# Autodesk Inventor assembly: Pass_Hang_subass
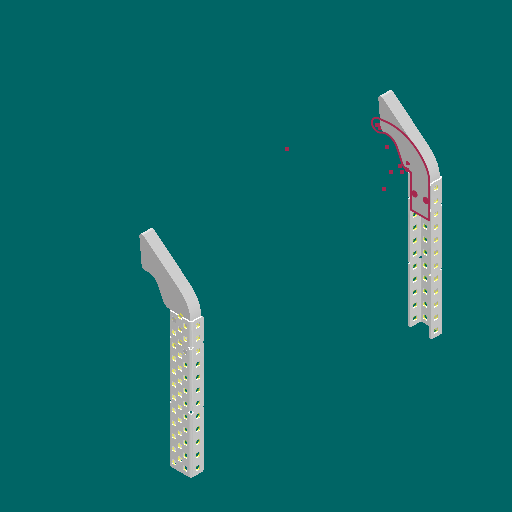
[picture p0: Inventor's stored thumbnail of the model, 512x512]
Saved by Autodesk Inventor 2025.2 (Build 292293000, 293)
## iProperties
Created: 2025-01-10
Part Number: Pass_Hang_subass
Document SubType Name: Assembly
Designer: Juanl
Author: Juanl
## Documents named in this file (4)
- C:\Users\colli\Documents\GitHub\ATUM-V5RC-High-Stakes-CAD\Robot\Subassemblies\Pass_Hang_subass.iam
- C:\Users\colli\Documents\GitHub\ATUM-V5RC-High-Stakes-CAD\Protobot\Pass_Hang_Hook.ipt
- C:\Users\colli\Documents\GitHub\ATUM-V5RC-High-Stakes-CAD\Protobot\Pass_Hang_Hook_MIR.ipt
- C:\Users\colli\Documents\GitHub\ATUM-V5RC-High-Stakes-CAD\VEX-CAD-Inventor\Structure\C Channel\Aluminum 1x2x1\Alu C 1x2x1x12.ipt
## Components (4 placed, 3 different names)
1. Pass_Hang_Hook:1 — Mate:3, Mate:4, Mate:5
2. Pass_Hang_Hook_MIR:1 — Mate:1, Mate:2, Mate:5
3. Alu C 1x2x1x12:2 — Flush:1, Mate:3, Mate:4, Mate:6
4. Alu C 1x2x1x12:1 — Flush:1, Mate:1, Mate:2, Mate:6
## Relationships (7: Mate 6, Flush 1)
- Flush:1: Alu C 1x2x1x12:2 ↔ Alu C 1x2x1x12:1
- Mate:1: Pass_Hang_Hook_MIR:1 ↔ Alu C 1x2x1x12:1
- Mate:2: Pass_Hang_Hook_MIR:1 ↔ Alu C 1x2x1x12:1
- Mate:3: Pass_Hang_Hook:1 ↔ Alu C 1x2x1x12:2
- Mate:4: Pass_Hang_Hook:1 ↔ Alu C 1x2x1x12:2
- Mate:5: Pass_Hang_Hook:1 ↔ Pass_Hang_Hook_MIR:1
- Mate:6 (282.5496 mm): Alu C 1x2x1x12:2 ↔ Alu C 1x2x1x12:1
